# Autodesk Inventor assembly: CuttingHead
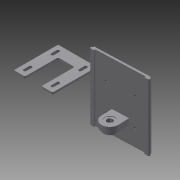
[picture p0: Inventor's stored thumbnail of the model, 180x180]
Saved by Autodesk Inventor 2013 (Build 170138000, 138)
## iProperties
Created: 2012-12-07
Part Number: CuttingHead
Document SubType Name: Assembly
Designer: istvan.burbank
Author: istvan.burbank
## Documents named in this file (7)
- D:\GitHub\Crown-Fire\CAD\Frame\CuttingHead\CuttingHead.iam
- D:\GitHub\Crown-Fire\CAD\Frame\CuttingHead\AcmeRoundNut.ipt
- D:\GitHub\Crown-Fire\CAD\Frame\CuttingHead\AcmeMountingFlange.ipt
- D:\GitHub\Crown-Fire\CAD\Frame\CuttingHead\backPlate.ipt
- D:\GitHub\Crown-Fire\CAD\Frame\CuttingHead\vee-track.ipt
- D:\GitHub\Crown-Fire\CAD\Templates\vee-track.ipt
- D:\GitHub\Crown-Fire\CAD\Frame\CuttingHead\torchMount_back.ipt
## Components (6 placed, 5 different names)
1. AcmeRoundNut:1 — Mate:1, Mate:2
2. AcmeMountingFlange:1 — Mate:1, Mate:2, Mate:3, Flush:3
3. backPlate:1 — Mate:3, Mate:4, Mate:5, Mate:6, Mate:7, Flush:1, Flush:2, Flush:3
4. vee-track:1 — Mate:4, Mate:7, Flush:1
5. vee-track:2 — Mate:5, Mate:6, Flush:2
6. torchMount_back:1
## Relationships (10: Mate 7, Flush 3)
- Mate:1: AcmeRoundNut:1 ↔ AcmeMountingFlange:1
- Mate:2: AcmeRoundNut:1 ↔ AcmeMountingFlange:1
- Mate:3: AcmeMountingFlange:1 ↔ backPlate:1
- Mate:4: backPlate:1 ↔ vee-track:1
- Mate:5: backPlate:1 ↔ vee-track:2
- Mate:6: backPlate:1 ↔ vee-track:2
- Mate:7: backPlate:1 ↔ vee-track:1
- Flush:1: backPlate:1 ↔ vee-track:1
- Flush:2: backPlate:1 ↔ vee-track:2
- Flush:3 (-38.1 mm): AcmeMountingFlange:1 ↔ backPlate:1
